# Autodesk Inventor assembly: 同步皮带传送
Saved by Autodesk Inventor 2015 (Build 190159000, 159)
## iProperties
Created: 2017-05-28
Part Number: 同步皮带传送
Document SubType Name: Assembly
Designer: Administrator
ClientObjectVersion: 1
Author: Administrator
## Documents named in this file (5)
- C:\Users\Administrator\Desktop\毕设改\总装配\设计加速器\同步皮带传送1.iam
- C:\Users\Administrator\Desktop\毕设改\总装配\设计加速器\同步皮带1.ipt
- C:\Users\Administrator\Desktop\毕设改\总装配\设计加速器\同步皮带轮11.ipt
- C:\Users\Administrator\Desktop\毕设改\总装配\设计加速器\同步皮带轮21.ipt
- C:\Users\Administrator\Desktop\毕设改\总装配\设计加速器\同步皮带轮31.ipt
## Components (4 placed, 4 different names)
1. 同步皮带:1 — 表面齐平:1, 配合:1, 配合:2, 表面齐平:2, 配合:3, 配合:4, 表面齐平:3, 配合:5, 配合:6
2. 同步皮带轮1:1 — 表面齐平:1, 配合:1, 配合:2, 转动:1, 转动:2
3. 同步皮带轮2:1 — 表面齐平:2, 配合:3, 转动:1, 配合:4
4. 同步皮带轮3:1 — 表面齐平:3, 配合:5, 转动:2, 配合:6
## Relationships (11: Mate 6, Flush 3, RelateRotation 2)
- 表面齐平:1 [Flush]: 同步皮带:1 ↔ 同步皮带轮1:1
- 配合:1 [Mate]: 同步皮带:1 ↔ 同步皮带轮1:1
- 配合:2 [Mate]: 同步皮带:1 ↔ 同步皮带轮1:1
- 表面齐平:2 [Flush]: 同步皮带:1 ↔ 同步皮带轮2:1
- 配合:3 [Mate]: 同步皮带:1 ↔ 同步皮带轮2:1
- 转动:1 [RelateRotation] (4 ul): 同步皮带轮1:1 ↔ 同步皮带轮2:1
- 配合:4 [Mate]: 同步皮带:1 ↔ 同步皮带轮2:1
- 表面齐平:3 [Flush]: 同步皮带:1 ↔ 同步皮带轮3:1
- 配合:5 [Mate]: 同步皮带:1 ↔ 同步皮带轮3:1
- 转动:2 [RelateRotation] (1 ul): 同步皮带轮1:1 ↔ 同步皮带轮3:1
- 配合:6 [Mate]: 同步皮带:1 ↔ 同步皮带轮3:1
